# Autodesk Inventor assembly: PCB enclosure_v3
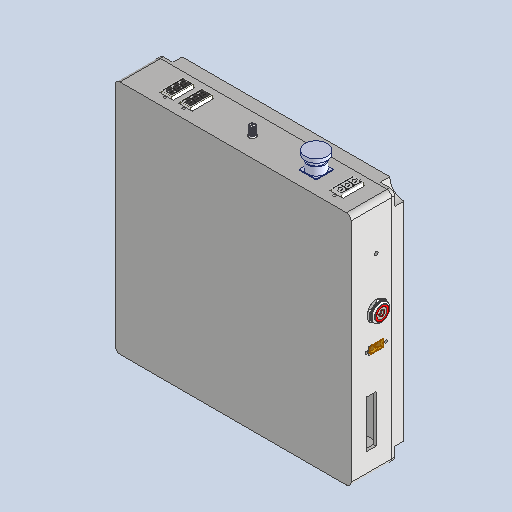
[picture p0: Inventor's stored thumbnail of the model, 512x512]
Saved by Autodesk Inventor 2026 (Build 300175050, 175E)
## iProperties
Created: 2025-10-28
Part Number: PCB enclosure_v3
Document SubType Name: Assembly
Designer: Kartik
Mass: 734.445 g
Surface Area: 6378.6 cm^2
Volume: 703.986 cm^3
Density: 1.04327 g/cm^3
Author: Kartik
## iProperties of the stored document KF350-3P v1 (2)_1.iam
Part Number: KF350-3P v1 (2)_1
Document SubType Name: Assembly
Designer: Kartik
Mass: 1.57749 g
Surface Area: 11.0557 cm^2
Volume: 0.464258 cm^3
Density: 3.39786 g/cm^3
Author: Kartik
## iProperties of the stored document Arduino Uno Screw Shield.iam
Created: 2019-11-19
Part Number: Arduino Uno Screw Shield
Document SubType Name: Assembly
Designer: Kartik
Mass: 41.3566 g
Surface Area: 261.032 cm^2
Volume: 12.8673 cm^3
Density: 3.21409 g/cm^3
Sending System: Autodesk Translation Framework v8.12.0.6
Preprocessor: ST-DEVELOPER v18
Title: C:/Users/ivano/Desktop/Arduino Uno Screw Shield v3.step
## iProperties of the stored document Stiftleiste_Male v3 (2).ipt
Part Number: Stiftleiste_Male v3 (2)
Material: Steel
Document SubType Name: Modeling
Designer: Kartik
Mass: 0.147893 g
Surface Area: 0.565392 cm^2
Volume: 0.0188399 cm^3
Density: 7.85 g/cm^3
Appearance: Default
Author: Kartik
## iProperties of the stored document KF350-2P v2.iam
Part Number: KF350-2P v2
Document SubType Name: Assembly
Designer: Kartik
Mass: 1.05166 g
Surface Area: 7.73072 cm^2
Volume: 0.309506 cm^3
Density: 3.39786 g/cm^3
Author: Kartik
## iProperties of the stored document Stiftleiste_Male v3.ipt
Part Number: Stiftleiste_Male v3
Material: Steel
Document SubType Name: Modeling
Designer: Kartik
Mass: 0.147893 g
Surface Area: 0.565392 cm^2
Volume: 0.0188399 cm^3
Density: 7.85 g/cm^3
Appearance: Default
Author: Kartik
## iProperties of the stored document KF350-3P v1.iam
Part Number: KF350-3P v1
Document SubType Name: Assembly
Designer: Kartik
Mass: 1.57749 g
Surface Area: 11.0557 cm^2
Volume: 0.464258 cm^3
Density: 3.39786 g/cm^3
Author: Kartik
## iProperties of the stored document Housing.ipt
Part Number: Housing
Material: ABS Plastic
Document SubType Name: Modeling
Designer: Kartik
Mass: 0.322674 g
Surface Area: 6.93271 cm^2
Volume: 0.30441 cm^3
Density: 1.06 g/cm^3
Appearance: Default
Author: Kartik
## iProperties of the stored document KF350-3P v1_2.iam
Part Number: KF350-3P v1_2
Document SubType Name: Assembly
Designer: Kartik
Mass: 1.57749 g
Surface Area: 11.0557 cm^2
Volume: 0.464258 cm^3
Density: 3.39786 g/cm^3
Author: Kartik
## iProperties of the stored document Contact Pin (3).ipt
Part Number: Contact Pin (3)
Material: Steel
Document SubType Name: Modeling
Designer: Kartik
Mass: 0.41827 g
Surface Area: 1.37432 cm^2
Volume: 0.0532829 cm^3
Density: 7.85 g/cm^3
Appearance: Default
Author: Kartik
## iProperties of the stored document KF350-3P v1 (2).iam
Part Number: KF350-3P v1 (2)
Document SubType Name: Assembly
Designer: Kartik
Mass: 1.57749 g
Surface Area: 11.0557 cm^2
Volume: 0.464258 cm^3
Density: 3.39786 g/cm^3
Author: Kartik
## iProperties of the stored document Tactile_SMD_3x6x2.5mm v3.ipt
Part Number: Tactile_SMD_3x6x2.5mm v3
Material: Steel
Document SubType Name: Modeling
Designer: Kartik
Mass: 0.310161 g
Surface Area: 0.834739 cm^2
Volume: 0.0395109 cm^3
Density: 7.85 g/cm^3
Appearance: Default
Author: Kartik
## iProperties of the stored document KF350-3P v1_3.iam
Part Number: KF350-3P v1_3
Document SubType Name: Assembly
Designer: Kartik
Mass: 1.57749 g
Surface Area: 11.0557 cm^2
Volume: 0.464258 cm^3
Density: 3.39786 g/cm^3
Author: Kartik
## iProperties of the stored document Buchsenleiste_female v2.ipt
Part Number: Buchsenleiste_female v2
Material: Steel
Document SubType Name: Modeling
Designer: Kartik
Mass: 0.378315 g
Surface Area: 1.18228 cm^2
Volume: 0.0481929 cm^3
Density: 7.85 g/cm^3
Appearance: Default
Author: Kartik
## iProperties of the stored document Housing (3).ipt
Part Number: Housing (3)
Material: ABS Plastic
Document SubType Name: Modeling
Designer: Kartik
Mass: 0.322674 g
Surface Area: 6.93271 cm^2
Volume: 0.30441 cm^3
Density: 1.06 g/cm^3
Appearance: Default
Author: Kartik
## iProperties of the stored document Stiftleiste_Male v3 (1).ipt
Part Number: Stiftleiste_Male v3 (1)
Material: Steel
Document SubType Name: Modeling
Designer: Kartik
Mass: 0.147893 g
Surface Area: 0.565392 cm^2
Volume: 0.0188399 cm^3
Density: 7.85 g/cm^3
Appearance: Default
Author: Kartik
## iProperties of the stored document PCB v19.ipt
Part Number: PCB v19
Material: GFRP
Document SubType Name: Modeling
Designer: Kartik
Mass: 11.5787 g
Surface Area: 107.169 cm^2
Volume: 6.61641 cm^3
Density: 1.75 g/cm^3
Appearance: Default
Author: Kartik
## iProperties of the stored document Housing (2).ipt
Part Number: Housing (2)
Material: ABS Plastic
Document SubType Name: Modeling
Designer: Kartik
Mass: 0.215116 g
Surface Area: 4.98207 cm^2
Volume: 0.20294 cm^3
Density: 1.06 g/cm^3
Appearance: Default
Author: Kartik
## iProperties of the stored document Contact Pin (2).ipt
Part Number: Contact Pin (2)
Material: Steel
Document SubType Name: Modeling
Designer: Kartik
Mass: 0.41827 g
Surface Area: 1.37432 cm^2
Volume: 0.0532829 cm^3
Density: 7.85 g/cm^3
Appearance: Default
Author: Kartik
## iProperties of the stored document KF350-3P v1 (1)_1.iam
Part Number: KF350-3P v1 (1)_1
Document SubType Name: Assembly
Designer: Kartik
Mass: 1.57749 g
Surface Area: 11.0557 cm^2
Volume: 0.464258 cm^3
Density: 3.39786 g/cm^3
Author: Kartik
## iProperties of the stored document 0603 Chip SMD LED (1.6x0.8mm) v2.ipt
Part Number: 0603 Chip SMD LED (1.6x0.8mm) v2
Material: Steel
Document SubType Name: Modeling
Designer: Kartik
Mass: 0.00549825 g
Surface Area: 0.105939 cm^2
Volume: 0.000700413 cm^3
Density: 7.85 g/cm^3
Appearance: Default
Author: Kartik
## iProperties of the stored document KF350-3P v1_1.iam
Part Number: KF350-3P v1_1
Document SubType Name: Assembly
Designer: Kartik
Mass: 1.57749 g
Surface Area: 11.0557 cm^2
Volume: 0.464258 cm^3
Density: 3.39786 g/cm^3
Author: Kartik
## iProperties of the stored document Contact Pin (1).ipt
Part Number: Contact Pin (1)
Material: Steel
Document SubType Name: Modeling
Designer: Kartik
Mass: 0.41827 g
Surface Area: 1.37432 cm^2
Volume: 0.0532829 cm^3
Density: 7.85 g/cm^3
Appearance: Default
Author: Kartik
## iProperties of the stored document KF350-2P v2_1.iam
Part Number: KF350-2P v2_1
Document SubType Name: Assembly
Designer: Kartik
Mass: 1.05166 g
Surface Area: 7.73072 cm^2
Volume: 0.309506 cm^3
Density: 3.39786 g/cm^3
Author: Kartik
## iProperties of the stored document Resistor 0603 v1.ipt
Part Number: Resistor 0603 v1
Material: Steel
Document SubType Name: Modeling
Designer: Kartik
Mass: 0.00520856 g
Surface Area: 0.0814478 cm^2
Volume: 0.00066351 cm^3
Density: 7.85 g/cm^3
Appearance: Default
Author: Kartik
## iProperties of the stored document Buchsenleiste_female v2 (2).ipt
Part Number: Buchsenleiste_female v2 (2)
Material: Steel
Document SubType Name: Modeling
Designer: Kartik
Mass: 0.378315 g
Surface Area: 1.18228 cm^2
Volume: 0.0481929 cm^3
Density: 7.85 g/cm^3
Appearance: Default
Author: Kartik
## iProperties of the stored document Contact Pin.ipt
Part Number: Contact Pin
Material: Steel
Document SubType Name: Modeling
Designer: Kartik
Mass: 0.41827 g
Surface Area: 1.37432 cm^2
Volume: 0.0532829 cm^3
Density: 7.85 g/cm^3
Appearance: Default
Author: Kartik
## iProperties of the stored document Buchsenleiste_female v2 (1).ipt
Part Number: Buchsenleiste_female v2 (1)
Material: Steel
Document SubType Name: Modeling
Designer: Kartik
Mass: 0.378315 g
Surface Area: 1.18228 cm^2
Volume: 0.0481929 cm^3
Density: 7.85 g/cm^3
Appearance: Default
Author: Kartik
## iProperties of the stored document KF350-3P v1 (1).iam
Part Number: KF350-3P v1 (1)
Document SubType Name: Assembly
Designer: Kartik
Mass: 1.57749 g
Surface Area: 11.0557 cm^2
Volume: 0.464258 cm^3
Density: 3.39786 g/cm^3
Author: Kartik
## iProperties of the stored document Housing (1).ipt
Part Number: Housing (1)
Material: ABS Plastic
Document SubType Name: Modeling
Designer: Kartik
Mass: 0.322674 g
Surface Area: 6.93271 cm^2
Volume: 0.30441 cm^3
Density: 1.06 g/cm^3
Appearance: Default
Author: Kartik
## Documents named in this file (46)
- D:\Kartik\Projects\AMR\CAD\2 Sub-assembly\PCB enclosure_v3.iam
- D:\Kartik\Projects\AMR\CAD\4 Boughtouts\MDD20A CAD\MDD20A\MDD20A\MDD20A.ipt
- D:\Kartik\Projects\AMR\CAD\4 Boughtouts\NUCLEO-F401RE--3DModel-STEP-56544\NUCLEO-F401RE--3DModel-STEP-56544\NUCLEO-F401RE--3DModel-STEP-56544.ipt
- D:\Kartik\Projects\AMR\CAD\4 Boughtouts\nvidia-jetson-nano-4gb\Jetson nano 4GB\Jetson nano 4GB\Jetson nano 4GB.ipt
- D:\Kartik\Projects\AMR\CAD\4 Boughtouts\arduino-uno-screw-shield-1\Arduino Uno Screw Shield\Arduino Uno Screw Shield\Arduino Uno Screw Shield.ipt
- D:\Kartik\Projects\AMR\CAD\4 Boughtouts\xh-m401-buck-converter\XH-M401 Buck converter (XL4016E1)\XH-M401 Buck converter (XL4016E1)\XH-M401 Buck converter (XL4016E1).ipt
- D:\Kartik\Projects\AMR\CAD\4 Boughtouts\LM2596 DC-DC StepDown Converter v1\LM2596 DC-DC StepDown Converter v1\LM2596 DC-DC StepDown Converter v1.ipt
- D:\Kartik\Projects\AMR\CAD\4 Boughtouts\push-button-16-mm-led-1\LED_Button16mm\LED_Button_16mm\LED_Button_16mm\LED_Button_16mm.ipt
- D:\Kartik\Projects\AMR\CAD\4 Boughtouts\electrical-part-fuse-holder\Fuse Holder - CONQUER CQ-201N_.iam
- D:\Kartik\Projects\AMR\CAD\4 Boughtouts\volt-meter-led-display-1\LED Display v3\LED Display v3\LED Display v3.ipt
- D:\Kartik\Projects\AMR\CAD\4 Boughtouts\volt-meter-led-display-1\LED Display v3\Amass XT60E1-M v4.ipt
- D:\Kartik\Projects\AMR\CAD\4 Boughtouts\mini-toggle-switches-1\6mm SPDT Mini Toggle Switch\6mm SPDT Mini Toggle Switch\6mm SPDT Mini Toggle Switch.ipt
- D:\Kartik\Projects\AMR\CAD\4 Boughtouts\emergency-stop-push-button-switches-ab6-v-series-16mm-1\AB6-V\AB6-V\AB6-V.ipt
- D:\Kartik\Projects\AMR\CAD\3 Parts\Enclosure_Plate.ipt
- D:\Kartik\Projects\AMR\CAD\3 Parts\current sensor.ipt
- **D:\Kartik\Projects\AMR\CAD\2 Sub-assembly\PCB enclosure_v3.iam*LocalDocs*xAaaaa4baAaaaaaaaAaaaat2yYg*Arduino Uno Screw Shield.iam
- D:\Kartik\Projects\AMR\CAD\3 Parts\Enclosure cover.ipt
- **D:\Kartik\Projects\AMR\CAD\2 Sub-assembly\PCB enclosure_v3.iam*LocalDocs*xAaaaafdaAaaaaaaaAaaaak3cDd*KF350-3P v1 (2)_1.iam
- **D:\Kartik\Projects\AMR\CAD\2 Sub-assembly\PCB enclosure_v3.iam*LocalDocs*xAaaaaqdaAaaaaaaaAaaaqd02Hd*Housing (3).ipt
- **D:\Kartik\Projects\AMR\CAD\2 Sub-assembly\PCB enclosure_v3.iam*LocalDocs*xAaaaaudaAaaaaaaaAaaaqnd5Bh*Contact Pin (3).ipt
- **D:\Kartik\Projects\AMR\CAD\2 Sub-assembly\PCB enclosure_v3.iam*LocalDocs*xAaaaarbaAaaaaaaaAaaaq1bhLa*PCB v19.ipt
- **D:\Kartik\Projects\AMR\CAD\2 Sub-assembly\PCB enclosure_v3.iam*LocalDocs*xAaaaa5caAaaaaaaaAaaaqmznWe*KF350-3P v1.iam
- **D:\Kartik\Projects\AMR\CAD\2 Sub-assembly\PCB enclosure_v3.iam*LocalDocs*xAaaaqqcaAaaaaaaaAaaaa22vYe*KF350-3P v1_1.iam
- **D:\Kartik\Projects\AMR\CAD\2 Sub-assembly\PCB enclosure_v3.iam*LocalDocs*xAaaaadcaAaaaaaaaAaaaqt1yTd*KF350-3P v1_2.iam
- **D:\Kartik\Projects\AMR\CAD\2 Sub-assembly\PCB enclosure_v3.iam*LocalDocs*xAaaaakbaAaaaaaaaAaaaq4jqKa*KF350-3P v1_3.iam
- **D:\Kartik\Projects\AMR\CAD\2 Sub-assembly\PCB enclosure_v3.iam*LocalDocs*xAaaaqycaAaaaaaaaAaaaqngf4h*KF350-3P v1 (1).iam
- **D:\Kartik\Projects\AMR\CAD\2 Sub-assembly\PCB enclosure_v3.iam*LocalDocs*xAaaaaybaAaaaaaaaAaaaqoddQg*KF350-3P v1 (1)_1.iam
- **D:\Kartik\Projects\AMR\CAD\2 Sub-assembly\PCB enclosure_v3.iam*LocalDocs*xAaaaa0caAaaaaaaaAaaaqc4aEd*KF350-2P v2.iam
- **D:\Kartik\Projects\AMR\CAD\2 Sub-assembly\PCB enclosure_v3.iam*LocalDocs*xAaaaqidaAaaaaaaaAaaaqzmdKb*KF350-2P v2_1.iam
- **D:\Kartik\Projects\AMR\CAD\2 Sub-assembly\PCB enclosure_v3.iam*LocalDocs*xAaaaamaaAaaaaaaaAaaaqz1mNf*KF350-3P v1 (2).iam
- **D:\Kartik\Projects\AMR\CAD\2 Sub-assembly\PCB enclosure_v3.iam*LocalDocs*xAaaaalcaAaaaaaaaAaaaqrc1Pd*Buchsenleiste_female v2.ipt
- **D:\Kartik\Projects\AMR\CAD\2 Sub-assembly\PCB enclosure_v3.iam*LocalDocs*xAaaaa3baAaaaaaaaAaaaq5phNd*Stiftleiste_Male v3.ipt
- **D:\Kartik\Projects\AMR\CAD\2 Sub-assembly\PCB enclosure_v3.iam*LocalDocs*xAaaaqzaaAaaaaaaaAaaaqy3xXf*Buchsenleiste_female v2 (1).ipt
- **D:\Kartik\Projects\AMR\CAD\2 Sub-assembly\PCB enclosure_v3.iam*LocalDocs*xAaaaaqcaAaaaaaaaAaaaafubVd*Stiftleiste_Male v3 (1).ipt
- **D:\Kartik\Projects\AMR\CAD\2 Sub-assembly\PCB enclosure_v3.iam*LocalDocs*xAaaaqxcaAaaaaaaaAaaaqkzqEe*Buchsenleiste_female v2 (2).ipt
- **D:\Kartik\Projects\AMR\CAD\2 Sub-assembly\PCB enclosure_v3.iam*LocalDocs*xAaaaa2daAaaaaaaaAaaaas50Gc*Stiftleiste_Male v3 (2).ipt
- **D:\Kartik\Projects\AMR\CAD\2 Sub-assembly\PCB enclosure_v3.iam*LocalDocs*xAaaaakdaAaaaaaaaAaaaak5t3b*Tactile_SMD_3x6x2.5mm v3.ipt
- **D:\Kartik\Projects\AMR\CAD\2 Sub-assembly\PCB enclosure_v3.iam*LocalDocs*xAaaaq3baAaaaaaaaAaaaqeazWh*0603 Chip SMD LED (1.6x0.8mm) v2.ipt
- **D:\Kartik\Projects\AMR\CAD\2 Sub-assembly\PCB enclosure_v3.iam*LocalDocs*xAaaaqobaAaaaaaaaAaaaqdouZf*Resistor 0603 v1.ipt
- **D:\Kartik\Projects\AMR\CAD\2 Sub-assembly\PCB enclosure_v3.iam*LocalDocs*xAaaaq3caAaaaaaaaAaaaadllWd*Housing (2).ipt
- **D:\Kartik\Projects\AMR\CAD\2 Sub-assembly\PCB enclosure_v3.iam*LocalDocs*xAaaaazaaAaaaaaaaAaaaa110Qe*Contact Pin (2).ipt
- **D:\Kartik\Projects\AMR\CAD\2 Sub-assembly\PCB enclosure_v3.iam*LocalDocs*xAaaaa4daAaaaaaaaAaaaa1hw3d*Housing.ipt
- **D:\Kartik\Projects\AMR\CAD\2 Sub-assembly\PCB enclosure_v3.iam*LocalDocs*xAaaaqvbaAaaaaaaaAaaaqhft1f*Contact Pin.ipt
- **D:\Kartik\Projects\AMR\CAD\2 Sub-assembly\PCB enclosure_v3.iam*LocalDocs*xAaaaqzaaAaaaaaaaAaaaqylcFd*Housing (1).ipt
- **D:\Kartik\Projects\AMR\CAD\2 Sub-assembly\PCB enclosure_v3.iam*LocalDocs*xAaaaqoaaAaaaaaaaAaaaqgtxDd*Contact Pin (1).ipt
- D:\Kartik\Projects\AMR\CAD\4 Boughtouts\arduino-uno-screw-shield-1\Arduino Uno Screw Shield.step
## Components (21 placed, 15 different names)
1. MDD20A:1 — Flush:11, Mate:28, Angle:3, Mate:69, Mate:70
2. NUCLEO-F401RE--3DModel-STEP-56544:1 — Mate:25, Mate:26, Mate:27, Mate:30, Angle:1, Mate:43, Mate:44, Mate:45, Mate:68
3. Jetson nano 4GB:1 — Mate:31, Angle:2, Mate:51, Mate:60
4. Arduino Uno Screw Shield:1 — Mate:25, Mate:26, Mate:27
5. XH-M401 Buck converter (XL4016E1):1 — Flush:11, Flush:19, Flush:20, Mate:66
6. LM2596 DC-DC StepDown Converter v1:1 — Mate:29, Mate:71, Mate:74
7. LED_Button_16mm:1 — Mate:38, Mate:49
8. Fuse Holder - CONQUER CQ-201N_:2 [sub-assembly] — Mate:35, Mate:52
9. LED Display v3:1 — Mate:54, Mate:55
10. Amass XT60E1-M v4:1 — Mate:46, Mate:47, Mate:48
11. 6mm SPDT Mini Toggle Switch:1 — Mate:37, Mate:76
12. AB6-V:1 — Mate:64, Mate:65
13. Enclosure_Plate:1 — Mate:28, Mate:29, Mate:30, Mate:31, Angle:1, Angle:2, Angle:3, Mate:32, Mate:33, Angle:4, Mate:35, Mate:37, Mate:38, Mate:46, Mate:47, Mate:48, Mate:49, Mate:51, Mate:52, Mate:53, Mate:54, Mate:55, Mate:56, Mate:57, Mate:58, Mate:59, Mate:60, Mate:64, Mate:65, Mate:66, Mate:67, Mate:68, Mate:69, Mate:70, Mate:71, Mate:72, Mate:73, Mate:74, Mate:75, Mate:76, Mate:77, Flush:21, Flush:22
14. current sensor:1 — Mate:32, Angle:5, Mate:72
15. current sensor:2 — Mate:33, Angle:4, Angle:5, Mate:73
16. XH-M401 Buck converter (XL4016E1):2 — Flush:19, Flush:20, Mate:67
17. LED Display v3:2 — Mate:56, Mate:59
18. LED Display v3:3 — Mate:57, Mate:58
19. Arduino Uno Screw Shield:2 [sub-assembly] — Mate:43, Mate:44, Mate:45
20. 6mm SPDT Mini Toggle Switch:2 — Mate:53, Mate:75
21. Enclosure cover:1 — Mate:77, Flush:21, Flush:22
## Relationships (53: Mate 43, Flush 5, Angle 5)
- Mate:25: NUCLEO-F401RE--3DModel-STEP-56544:1 ↔ Arduino Uno Screw Shield:1
- Mate:26: NUCLEO-F401RE--3DModel-STEP-56544:1 ↔ Arduino Uno Screw Shield:1
- Mate:27: NUCLEO-F401RE--3DModel-STEP-56544:1 ↔ Arduino Uno Screw Shield:1
- Flush:11: MDD20A:1 ↔ XH-M401 Buck converter (XL4016E1):1
- Mate:28 (10 mm): MDD20A:1 ↔ Enclosure_Plate:1
- Mate:29 (10 mm): LM2596 DC-DC StepDown Converter v1:1 ↔ Enclosure_Plate:1
- Mate:30 (10 mm): NUCLEO-F401RE--3DModel-STEP-56544:1 ↔ Enclosure_Plate:1
- Mate:31 (10 mm): Jetson nano 4GB:1 ↔ Enclosure_Plate:1
- Angle:1 (-90 deg): NUCLEO-F401RE--3DModel-STEP-56544:1 ↔ Enclosure_Plate:1
- Angle:2 (-90 deg): Jetson nano 4GB:1 ↔ Enclosure_Plate:1
- Angle:3 (0 deg): MDD20A:1 ↔ Enclosure_Plate:1
- Mate:32 (10 mm): Enclosure_Plate:1 ↔ current sensor:1
- Mate:33 (10 mm): Enclosure_Plate:1 ↔ current sensor:2
- Angle:4 (0 deg): Enclosure_Plate:1 ↔ current sensor:2
- Angle:5 (0 deg): current sensor:1 ↔ current sensor:2
- Mate:35: Fuse Holder - CONQUER CQ-201N_:2 ↔ Enclosure_Plate:1
- Mate:37: 6mm SPDT Mini Toggle Switch:1 ↔ Enclosure_Plate:1
- Flush:19: XH-M401 Buck converter (XL4016E1):1 ↔ XH-M401 Buck converter (XL4016E1):2
- Mate:38: LED_Button_16mm:1 ↔ Enclosure_Plate:1
- Mate:43: NUCLEO-F401RE--3DModel-STEP-56544:1 ↔ Arduino Uno Screw Shield:2
- Mate:44: NUCLEO-F401RE--3DModel-STEP-56544:1 ↔ Arduino Uno Screw Shield:2
- Mate:45: NUCLEO-F401RE--3DModel-STEP-56544:1 ↔ Arduino Uno Screw Shield:2
- Mate:46: Amass XT60E1-M v4:1 ↔ Enclosure_Plate:1
- Mate:47: Amass XT60E1-M v4:1 ↔ Enclosure_Plate:1
- Mate:48: Amass XT60E1-M v4:1 ↔ Enclosure_Plate:1
- Mate:49: LED_Button_16mm:1 ↔ Enclosure_Plate:1
- Mate:51 (0.1 mm): Jetson nano 4GB:1 ↔ Enclosure_Plate:1
- Mate:52: Fuse Holder - CONQUER CQ-201N_:2 ↔ Enclosure_Plate:1
- Mate:53: Enclosure_Plate:1 ↔ 6mm SPDT Mini Toggle Switch:2
- Mate:54: LED Display v3:1 ↔ Enclosure_Plate:1
- Mate:55: LED Display v3:1 ↔ Enclosure_Plate:1
- Mate:56: Enclosure_Plate:1 ↔ LED Display v3:2
- Mate:57: Enclosure_Plate:1 ↔ LED Display v3:3
- Mate:58: Enclosure_Plate:1 ↔ LED Display v3:3
- Mate:59: Enclosure_Plate:1 ↔ LED Display v3:2
- Mate:60 (20 mm): Jetson nano 4GB:1 ↔ Enclosure_Plate:1
- Flush:20: XH-M401 Buck converter (XL4016E1):1 ↔ XH-M401 Buck converter (XL4016E1):2
- Mate:64: AB6-V:1 ↔ Enclosure_Plate:1
- Mate:65: AB6-V:1 ↔ Enclosure_Plate:1
- Mate:66: XH-M401 Buck converter (XL4016E1):1 ↔ Enclosure_Plate:1
- Mate:67: Enclosure_Plate:1 ↔ XH-M401 Buck converter (XL4016E1):2
- Mate:68: NUCLEO-F401RE--3DModel-STEP-56544:1 ↔ Enclosure_Plate:1
- Mate:69 (-2.54 mm): MDD20A:1 ↔ Enclosure_Plate:1
- Mate:70 (-2.54 mm): MDD20A:1 ↔ Enclosure_Plate:1
- Mate:71: LM2596 DC-DC StepDown Converter v1:1 ↔ Enclosure_Plate:1
- Mate:72: Enclosure_Plate:1 ↔ current sensor:1
- Mate:73: Enclosure_Plate:1 ↔ current sensor:2
- Mate:74: LM2596 DC-DC StepDown Converter v1:1 ↔ Enclosure_Plate:1
- Mate:75: Enclosure_Plate:1 ↔ 6mm SPDT Mini Toggle Switch:2
- Mate:76: 6mm SPDT Mini Toggle Switch:1 ↔ Enclosure_Plate:1
- Mate:77: Enclosure_Plate:1 ↔ Enclosure cover:1
- Flush:21: Enclosure_Plate:1 ↔ Enclosure cover:1
- Flush:22: Enclosure_Plate:1 ↔ Enclosure cover:1
